# Autodesk Inventor assembly: AirPressureValve
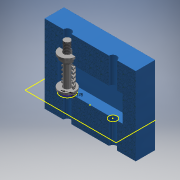
[picture p0: Inventor's stored thumbnail of the model, 180x180]
Saved by Autodesk Inventor 2018 (Build 220112000, 112)
## iProperties
Created: 2020-03-27
Part Number: AirPressureValve
Document SubType Name: Assembly
Designer: emile
Author: emile
## Documents named in this file (9)
- C:\Users\emile\OneDrive\Documents\Inventor\Respirator\Peep\AirPressureValve.iam
- C:\Users\emile\OneDrive\Documents\Inventor\Respirator\Peep\AirPressureAndValve.ipt
- C:\Users\emile\OneDrive\Documents\Inventor\Respirator\Peep\High-Temperature Silicone O-Ring(1283N198).ipt
- C:\Users\emile\OneDrive\Documents\Inventor\Respirator\Peep\AirPressureAndValvePart2.ipt
- C:\Users\emile\OneDrive\Documents\Inventor\Respirator\Peep\57785K110_FOOD-GRADE DRY-RUNNING SLEEVE BEARING.ipt
- C:\Users\emile\OneDrive\Documents\Inventor\Content Center Files\R2018\en-US\ANSI B18.5(05)\ANSI B18.5 - 1_4-20 UNC - 1.625(6).ipt
- C:\Users\emile\OneDrive\Documents\Inventor\Content Center Files\R2018\en-US\ANSI B18.2.2(08)\ANSI B18.2.2 - 1_4 - 20(3).ipt
- C:\Users\emile\OneDrive\Documents\Inventor\Content Center Files\R2018\en-US\ASTM F436(1)\ASTM F436 - 1_4(1).ipt
- C:\Users\emile\OneDrive\Documents\Inventor\Respirator\Peep\9001T270_PRECISION  SPRING.ipt
## Components (9 placed, 8 different names)
1. AirPressureAndValve:1 — Flush:1, Flush:2, Flush:3, Mate:1, Tangent:1, Mate:5, Mate:7
2. High-Temperature Silicone O-Ring(1283N198):1 — Mate:1, Tangent:1, Mate:6, Tangent:2
3. AirPressureAndValvePart2:1 — Mate:2, Mate:3, Mate:4, Mate:5, Mate:7
4. 57785K110_FOOD-GRADE DRY-RUNNING SLEEVE BEARING:1 — Mate:2, Mate:3
5. Round Head Bolt - Inch 1/4-20 UNC - 1.625:1 — Mate:4, Mate:6, Tangent:2, Mate:9, Mate:11, Mate:13, Mate:14, Mate:16
6. Hex Jam Nut - Inch 1/4 - 20:1 — Mate:9, Mate:12
7. Circular Washer (Inch) 1/4:1 — Mate:11, Mate:12
8. 9001T270_PRECISION  SPRING:1 — Mate:15, Mate:16
9. Circular Washer (Inch) 1/4:2 — Mate:13, Mate:14, Mate:15
## Relationships (19: Mate 14, Flush 3, Tangent 2)
- Flush:1: AirPressureAndValve:1
- Flush:2: AirPressureAndValve:1
- Flush:3: AirPressureAndValve:1
- Mate:1: AirPressureAndValve:1 ↔ High-Temperature Silicone O-Ring(1283N198):1
- Tangent:1: AirPressureAndValve:1 ↔ High-Temperature Silicone O-Ring(1283N198):1
- Mate:2: AirPressureAndValvePart2:1 ↔ 57785K110_FOOD-GRADE DRY-RUNNING SLEEVE BEARING:1
- Mate:3: AirPressureAndValvePart2:1 ↔ 57785K110_FOOD-GRADE DRY-RUNNING SLEEVE BEARING:1
- Mate:4: AirPressureAndValvePart2:1 ↔ Round Head Bolt - Inch 1/4-20 UNC - 1.625:1
- Mate:5: AirPressureAndValve:1 ↔ AirPressureAndValvePart2:1
- Mate:6: High-Temperature Silicone O-Ring(1283N198):1 ↔ Round Head Bolt - Inch 1/4-20 UNC - 1.625:1
- Tangent:2: High-Temperature Silicone O-Ring(1283N198):1 ↔ Round Head Bolt - Inch 1/4-20 UNC - 1.625:1
- Mate:7: AirPressureAndValve:1 ↔ AirPressureAndValvePart2:1
- Mate:9: Round Head Bolt - Inch 1/4-20 UNC - 1.625:1 ↔ Hex Jam Nut - Inch 1/4 - 20:1
- Mate:11: Round Head Bolt - Inch 1/4-20 UNC - 1.625:1 ↔ Circular Washer (Inch) 1/4:1
- Mate:12: Hex Jam Nut - Inch 1/4 - 20:1 ↔ Circular Washer (Inch) 1/4:1
- Mate:13: Round Head Bolt - Inch 1/4-20 UNC - 1.625:1 ↔ Circular Washer (Inch) 1/4:2
- Mate:14: Round Head Bolt - Inch 1/4-20 UNC - 1.625:1 ↔ Circular Washer (Inch) 1/4:2
- Mate:15: 9001T270_PRECISION  SPRING:1 ↔ Circular Washer (Inch) 1/4:2
- Mate:16: Round Head Bolt - Inch 1/4-20 UNC - 1.625:1 ↔ 9001T270_PRECISION  SPRING:1
